# Autodesk Inventor assembly: Extruder Carriage
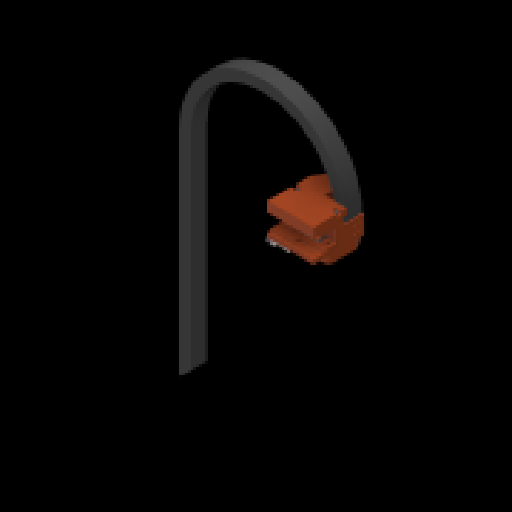
[picture p0: Inventor's stored thumbnail of the model, 512x512]
Saved by Autodesk Inventor 2023.3 (Build 273359000, 359)
## iProperties
Created: 2023-02-03
Part Number: Extruder Carriage
Document SubType Name: Assembly
Designer: remop
Author: remop
## Documents named in this file (15)
- C:\Users\remop\OneDrive\Documents\Inventor\3D Printers\LuEVO\Mk5_FullKinematic\XY Motion System\Extruder Carriage.iam
- C:\Users\remop\OneDrive\Documents\Inventor\3D Printers\LuEVO\Mk5_FullKinematic\XY Motion System\MGN12C.ipt
- C:\Users\remop\OneDrive\Documents\Inventor\3D Printers\LuEVO\Mk5_FullKinematic\XY Motion System\Toolhead\final_Toolhead.iam
- C:\Users\remop\OneDrive\Documents\Inventor\3D Printers\LuEVO\Mk5_FullKinematic\XY Motion System\Toolhead\Toolhead Base.ipt
- C:\Users\remop\OneDrive\Documents\Inventor\Content Center Files\R2023\en-US\AS 1427(04)\AS 1427 - M5 x 16(5) I.ipt
- C:\Users\remop\OneDrive\Documents\Inventor\Content Center Files\R2023\en-US\AS 1420\AS 1420 - 1973 - M3 x 8.ipt
- C:\Users\remop\OneDrive\Documents\Inventor\3D Printers\LuEVO\Mk5_FullKinematic\Electronics\Mellow Fly SHT36.ipt
- C:\Users\remop\OneDrive\Documents\Inventor\Content Center Files\R2023\en-US\AS 1427(05)\AS 1427 - M3 x 5(5) II.ipt
- C:\Users\remop\OneDrive\Documents\Inventor\3D Printers\LuEVO\Mk5_FullKinematic\XY Motion System\Toolhead\Drag Chain Base.ipt
- C:\Users\remop\OneDrive\Documents\Inventor\3D Printers\LuEVO\Mk5_FullKinematic\XY Motion System\Drag Chain Dummy.ipt
- C:\Users\remop\OneDrive\Documents\Inventor\3D Printers\LuEVO\Mk5_FullKinematic\Electronics\Nozzle Cam\Nozzlecam_PCB_Mount.ipt
- C:\Users\remop\OneDrive\Documents\Inventor\Content Center Files\R2023\en-US\ANSI B18.3.1M(6)\ANSI B18.3.1M - M1.6x0.35 x 5(1).ipt
- C:\Users\remop\OneDrive\Documents\Inventor\3D Printers\LuEVO\Mk5_FullKinematic\Electronics\PCB Endstop.ipt
- C:\Users\remop\OneDrive\Documents\Inventor\Content Center Files\R2023\en-US\DIN 7984\DIN 7984 - M3 x 5.ipt
- C:\Users\remop\OneDrive\Documents\Inventor\3D Printers\LuEVO\Mk5_FullKinematic\XY Motion System\Toolhead\Extruder Cover.ipt
## Components (28 placed, 14 different names)
1. MGN12C:1 — Mate:1, Mate:2, Flush:1
2. final_Toolhead:1 [sub-assembly] — Mate:1, Mate:2, Flush:1, Flush:2, Rotational:1, Rotational:2, Mate:5
3. Toolhead Base:1 — Flush:2, Flush:3, Mate:3, Flush:4, Flush:5, Flush:7, Rigid:1, Flush:10, Mate:6, Flush:11
4. AS 1427 H - Metric M5 x 16:1 — Rotational:2
5. AS 1427 H - Metric M5 x 16:2 — Rotational:1
6. AS 1420 - Metric M3 x 8:1
7. AS 1420 - Metric M3 x 8:2
8. AS 1420 - Metric M3 x 8:3
9. Mellow Fly SHT36:1 — Flush:3, Mate:3, Flush:4, Insert:4, Insert:5
10. AS 1427 H - Metric M3 x 5:1 — Insert:4
11. AS 1427 H - Metric M3 x 5:2 — Insert:5
12. Drag Chain Base:1 — Flush:5, Insert:6, Insert:7, Flush:6, Mate:4, Flush:8, Flush:9
13. AS 1420 - Metric M3 x 8:4 — Insert:6
14. AS 1420 - Metric M3 x 8:5 — Insert:7
15. Drag Chain Dummy:1 — Flush:6, Mate:4, Flush:8, Flush:9
16. Nozzlecam_PCB_Mount:1 — Flush:7, Rigid:1, Insert:8, Insert:9
17. AS 1420 - Metric M3 x 8:6 — Insert:8
18. AS 1420 - Metric M3 x 8:7 — Insert:9
19. Forged Socket Head Cap Screw - Metric M1.6x0.35 x 5:1
20. Forged Socket Head Cap Screw - Metric M1.6x0.35 x 5:2
21. Forged Socket Head Cap Screw - Metric M1.6x0.35 x 5:3
22. Forged Socket Head Cap Screw - Metric M1.6x0.35 x 5:4
23. PCB Endstop:1 — Mate:5, Flush:10, Mate:6, Insert:14, Insert:15
24. DIN 7984 M3 x 5:1 — Insert:14
25. DIN 7984 M3 x 5:2 — Insert:15
26. Extruder Cover:1 — Flush:11, Insert:16, Insert:17
27. AS 1420 - Metric M3 x 8:8 — Insert:16
28. AS 1420 - Metric M3 x 8:9 — Insert:17
## Relationships (30: Flush 11, Insert 10, Mate 6, RevoluteJoint 2, WeldJoint 1)
- Mate:1 (4 mm): MGN12C:1 ↔ final_Toolhead:1
- Mate:2 (-12 mm): MGN12C:1 ↔ final_Toolhead:1
- Flush:1 (13.795 mm): MGN12C:1 ↔ final_Toolhead:1
- Flush:2: final_Toolhead:1 ↔ Toolhead Base:1
- Rotational:1 [RevoluteJoint]: final_Toolhead:1 ↔ AS 1427 H - Metric M5 x 16:2
- Rotational:2 [RevoluteJoint]: final_Toolhead:1 ↔ AS 1427 H - Metric M5 x 16:1
- Flush:3 (5 mm): Toolhead Base:1 ↔ Mellow Fly SHT36:1
- Mate:3 (3 mm): Toolhead Base:1 ↔ Mellow Fly SHT36:1
- Flush:4 (5.365 mm): Toolhead Base:1 ↔ Mellow Fly SHT36:1
- Insert:4: Mellow Fly SHT36:1 ↔ AS 1427 H - Metric M3 x 5:1
- Insert:5: Mellow Fly SHT36:1 ↔ AS 1427 H - Metric M3 x 5:2
- Flush:5: Toolhead Base:1 ↔ Drag Chain Base:1
- Insert:6: Drag Chain Base:1 ↔ AS 1420 - Metric M3 x 8:4
- Insert:7: Drag Chain Base:1 ↔ AS 1420 - Metric M3 x 8:5
- Flush:6: Drag Chain Base:1 ↔ Drag Chain Dummy:1
- Flush:7: Toolhead Base:1 ↔ Nozzlecam_PCB_Mount:1
- Rigid:1 [WeldJoint]: Toolhead Base:1 ↔ Nozzlecam_PCB_Mount:1
- Insert:8: Nozzlecam_PCB_Mount:1 ↔ AS 1420 - Metric M3 x 8:6
- Insert:9: Nozzlecam_PCB_Mount:1 ↔ AS 1420 - Metric M3 x 8:7
- Mate:4: Drag Chain Base:1 ↔ Drag Chain Dummy:1
- Flush:8: Drag Chain Base:1 ↔ Drag Chain Dummy:1
- Flush:9 (5 mm): Drag Chain Base:1 ↔ Drag Chain Dummy:1
- Mate:5: final_Toolhead:1 ↔ PCB Endstop:1
- Flush:10 (1 mm): Toolhead Base:1 ↔ PCB Endstop:1
- Mate:6: Toolhead Base:1 ↔ PCB Endstop:1
- Insert:14: PCB Endstop:1 ↔ DIN 7984 M3 x 5:1
- Insert:15: PCB Endstop:1 ↔ DIN 7984 M3 x 5:2
- Flush:11: Toolhead Base:1 ↔ Extruder Cover:1
- Insert:16: Extruder Cover:1 ↔ AS 1420 - Metric M3 x 8:8
- Insert:17: Extruder Cover:1 ↔ AS 1420 - Metric M3 x 8:9
